# Autodesk Inventor assembly: 总装配
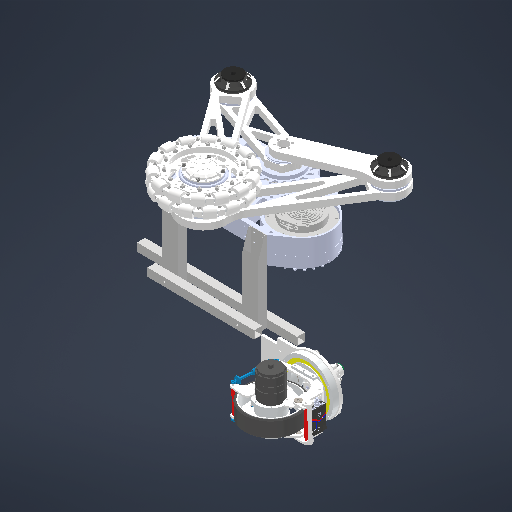
[picture p0: Inventor's stored thumbnail of the model, 512x512]
Saved by Autodesk Inventor 2025 (Build 290162000, 162)
## iProperties
Created: 2025-04-19
Part Number: 总装配
Document SubType Name: Assembly
Designer: XH
Author: XH
## Documents named in this file (8)
- C:\1A_Engineering_files\RCInventor\铝件版本\总装配.iam
- C:\1A_Engineering_files\RCInventor\铝件版本\GM6020 直流无刷电机_3.2.ipt
- C:\1A_Engineering_files\RCInventor\铝件版本\板材_云台连接板3.ipt
- C:\1A_Engineering_files\RCInventor\铝件版本\装配体2_MIR1.iam
- C:\1A_Engineering_files\RCInventor\铝件版本\铝方管\40x15_MIR.ipt
- C:\1A_Engineering_files\RCInventor\铝件版本\铝方管\15x15_MIR.ipt
- C:\1A_Engineering_files\RCInventor\铝件版本\铝方管\15x152.ipt
- C:\1A_Engineering_files\RCInventor\铝件版本\轮系\舵轮\RMDL2.0——00.iam
## Components (8 placed, 7 different names)
1. GM6020 直流无刷电机_3.2:1 — 配合:5, 配合:6, 配合:7
2. 板材_云台连接板3:1 — 配合:5, 配合:6, 配合:7
3. 装配体2_MIR1:1 [sub-assembly] — 表面齐平:7, 表面齐平:8, 配合:10, 配合:11, 表面齐平:9, 配合:12
4. 40x15_MIR:1 — 表面齐平:7, 表面齐平:8, 配合:10, 表面齐平:10, 配合:13, 配合:19
5. 40x15_MIR:2 — 配合:11, 表面齐平:9, 配合:12
6. 15x15_MIR:1 — 表面齐平:10, 配合:13, 配合:18, 配合:20, 配合:21
7. 15x152:2 — 配合:18, 配合:19, 配合:20
8. RMDL2.0——00:1 [sub-assembly] — 配合:21
## Relationships (16: Mate 11, Flush 5)
- 表面齐平:1 [Flush] (138 mm)
- 配合:5 [Mate]: GM6020 直流无刷电机_3.2:1 ↔ 板材_云台连接板3:1
- 配合:6 [Mate]: GM6020 直流无刷电机_3.2:1 ↔ 板材_云台连接板3:1
- 配合:7 [Mate]: GM6020 直流无刷电机_3.2:1 ↔ 板材_云台连接板3:1
- 表面齐平:7 [Flush]: 装配体2_MIR1:1 ↔ 40x15_MIR:1
- 表面齐平:8 [Flush]: 装配体2_MIR1:1 ↔ 40x15_MIR:1
- 配合:10 [Mate]: 装配体2_MIR1:1 ↔ 40x15_MIR:1
- 配合:11 [Mate]: 装配体2_MIR1:1 ↔ 40x15_MIR:2
- 表面齐平:9 [Flush]: 装配体2_MIR1:1 ↔ 40x15_MIR:2
- 配合:12 [Mate]: 装配体2_MIR1:1 ↔ 40x15_MIR:2
- 表面齐平:10 [Flush]: 40x15_MIR:1 ↔ 15x15_MIR:1
- 配合:13 [Mate]: 40x15_MIR:1 ↔ 15x15_MIR:1
- 配合:18 [Mate]: 15x15_MIR:1 ↔ 15x152:2
- 配合:19 [Mate]: 40x15_MIR:1 ↔ 15x152:2
- 配合:20 [Mate]: 15x15_MIR:1 ↔ 15x152:2
- 配合:21 [Mate]: 15x15_MIR:1 ↔ RMDL2.0——00:1
